# Autodesk Inventor assembly: HelixAssem
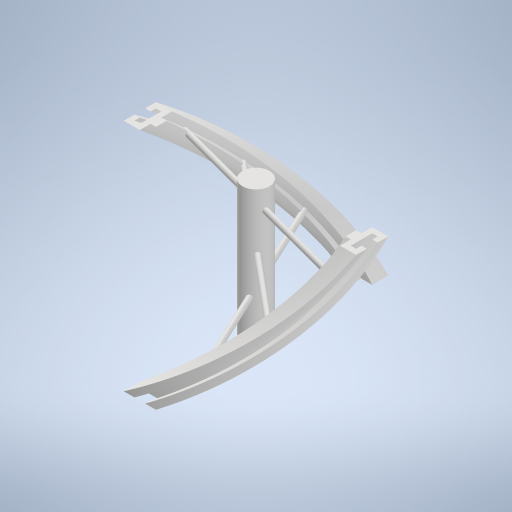
[picture p0: Inventor's stored thumbnail of the model, 512x512]
Saved by Autodesk Inventor 2023.2 (Build 272271000, 271)
## iProperties
Created: 2023-02-13
Part Number: HelixAssem
Document SubType Name: Assembly
Designer: atrus
Author: atrus
## Documents named in this file (3)
- C:\Users\atrus\Dropbox\elec\Mechanical\SkimmerSwabbie\HelixAssem.iam
- C:\Users\atrus\Dropbox\elec\Mechanical\SkimmerSwabbie\helix.ipt
- C:\Users\atrus\Dropbox\elec\Mechanical\SkimmerSwabbie\Brace.ipt
## Components (2 placed, 2 different names)
1. helix:1 — Flush:1
2. Brace:1 — Flush:1
## Relationships (1: Flush 1)
- Flush:1: helix:1 ↔ Brace:1
